# Autodesk Inventor assembly: Übertragung des Zahnriemens
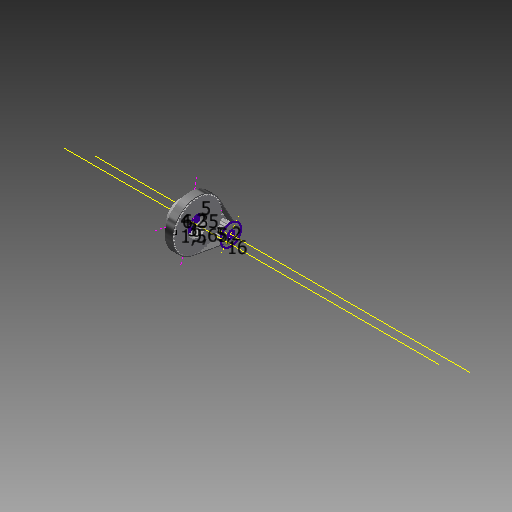
[picture p0: Inventor's stored thumbnail of the model, 512x512]
Saved by Autodesk Inventor 2018.3 (Build 223284000, 284)
## iProperties
Created: 2018-07-27
Part Number: Übertragung des Zahnriemens
Document SubType Name: Assembly
Designer: JochenAlt
ClientObjectVersion: 1
Author: JochenAlt
## Documents named in this file (4)
- D:\Projects\FlowerPot\CAD\Beltdrive\Konstruktions-Assistent\Übertragung des Zahnriemens2.iam
- D:\Projects\FlowerPot\CAD\Beltdrive\Konstruktions-Assistent\Zahnriemen2.ipt
- D:\Projects\FlowerPot\CAD\Beltdrive\Konstruktions-Assistent\Synchrone Riemenscheibe12.ipt
- D:\Projects\FlowerPot\CAD\Beltdrive\Konstruktions-Assistent\Synchrone Riemenscheibe22.ipt
## Components (3 placed, 3 different names)
1. Zahnriemen:1 — Fluchtend:1, Passend:1, Passend:2, Fluchtend:2, Passend:3, Passend:4
2. Synchrone Riemenscheibe1:1 — Fluchtend:1, Passend:1, Passend:2, Drehung:1
3. Synchrone Riemenscheibe2:1 — Fluchtend:2, Passend:3, Drehung:1, Passend:4
## Relationships (7: Mate 4, Flush 2, RelateRotation 1)
- Fluchtend:1 [Flush]: Zahnriemen:1 ↔ Synchrone Riemenscheibe1:1
- Passend:1 [Mate]: Zahnriemen:1 ↔ Synchrone Riemenscheibe1:1
- Passend:2 [Mate]: Zahnriemen:1 ↔ Synchrone Riemenscheibe1:1
- Fluchtend:2 [Flush]: Zahnriemen:1 ↔ Synchrone Riemenscheibe2:1
- Passend:3 [Mate]: Zahnriemen:1 ↔ Synchrone Riemenscheibe2:1
- Drehung:1 [RelateRotation] (3 ul): Synchrone Riemenscheibe1:1 ↔ Synchrone Riemenscheibe2:1
- Passend:4 [Mate]: Zahnriemen:1 ↔ Synchrone Riemenscheibe2:1
